# Autodesk Inventor assembly: Koło2
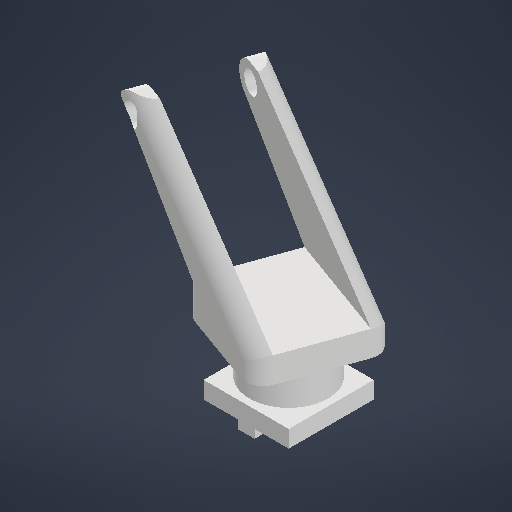
[picture p0: Inventor's stored thumbnail of the model, 512x512]
Saved by Autodesk Inventor 2026 (Build 300175000, 175)
## iProperties
Created: 2025-04-28
Part Number: Koło2
Document SubType Name: Assembly
Designer: isan
Author: isan
## Documents named in this file (5)
- E:\Conan II enhanced\Koło2.iam
- E:\Conan II enhanced\TrzymakNaLozysko.ipt
- E:\Conan II enhanced\Lozysko682ZZ.ipt
- E:\Conan II enhanced\RamaKola.ipt
- E:\Conan II enhanced\PodstawkaKola.ipt
## Components (4 placed, 4 different names)
1. TrzymakNaLozysko:1 — Mate:1, Mate:2, Mate:4
2. Lozysko682ZZ:1 — Mate:1, Mate:2, Mate:3
3. RamaKola:1 — Mate:3, Mate:4, Mate:5, Mate:6, Mate:7
4. PodstawkaKola:1 — Mate:5, Mate:6, Mate:7
## Relationships (7: Mate 7)
- Mate:1: TrzymakNaLozysko:1 ↔ Lozysko682ZZ:1
- Mate:2: TrzymakNaLozysko:1 ↔ Lozysko682ZZ:1
- Mate:3: Lozysko682ZZ:1 ↔ RamaKola:1
- Mate:4: TrzymakNaLozysko:1 ↔ RamaKola:1
- Mate:5: RamaKola:1 ↔ PodstawkaKola:1
- Mate:6 (0.2 mm): RamaKola:1 ↔ PodstawkaKola:1
- Mate:7 (-6.5 mm): RamaKola:1 ↔ PodstawkaKola:1
